# Autodesk Inventor assembly: Right Side Arm Intake
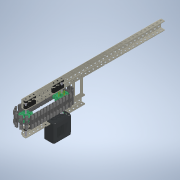
[picture p0: Inventor's stored thumbnail of the model, 180x180]
Saved by Autodesk Inventor 2020 (Build 240168000, 168)
## iProperties
Created: 2019-09-15
Part Number: Right Side Arm Intake
Document SubType Name: Assembly
Designer: Corey
Author: Corey
## Documents named in this file (10)
- C:\Users\Corey\Documents\Tower-Takeover-CAD\Parts\Right Side Arm Intake.iam
- C:\Users\Corey\Documents\Tower-Takeover-CAD\Parts\Motion\Sprockets\High Strength 12-tooth Sprocket.ipt
- C:\Users\Corey\Documents\Tower-Takeover-CAD\Parts\Structure\C-Channels\Aluminum\2-Wide\Aluminum C-Channel 1x2x1x35_MIR1.ipt
- C:\Users\Corey\Documents\Tower-Takeover-CAD\Parts\Motion\Bearing Flat_MIR4.ipt
- C:\Users\Corey\Documents\Tower-Takeover-CAD\Parts\Motion\Drive Shafts\Drive Shaft 4''_MIR1.ipt
- C:\Users\Corey\Documents\Tower-Takeover-CAD\Parts\Motion\Chain & Tank Tread\Tank Tread Traction Link_MIR1.ipt
- C:\Users\Corey\Documents\Tower-Takeover-CAD\Parts\Electronics\V5\Smart_Motor_MIR1.iam
- C:\Users\Corey\Documents\Tower-Takeover-CAD\Parts\Structure\Standoffs & Couplers\Standoff 2.00''_MIR1.ipt
- C:\Users\Corey\Documents\Tower-Takeover-CAD\Parts\Structure\C-Channels\Aluminum\2-Wide\Aluminum C-Channel 1x2x1x15_MIR1.ipt
- C:\Users\Corey\Documents\Tower-Takeover-CAD\Parts\Chain Sketch for Intake.ipt
## Components (51 placed, 9 different names)
1. Aluminum C-Channel 1x2x1x35_MIR1:1 — Insert:27, Insert:28, Mate:19, Insert:29, Insert:30, Mate:20, Insert:31, Insert:32, Mate:21, Insert:33, Insert:34, Mate:22, Insert:37, Insert:38, Mate:30, Mate:33
2. Bearing Flat_MIR4:1 — Insert:27, Insert:28, Mate:19
3. Bearing Flat_MIR4:2 — Insert:29, Insert:30, Mate:20, Insert:36
4. Bearing Flat_MIR4:3 — Insert:31, Insert:32, Mate:21
5. Bearing Flat_MIR4:4 — Insert:33, Insert:34, Mate:22, Insert:35
6. Drive Shaft 4''_MIR1:1 — Insert:35, Mate:31, Mate:32
7. Drive Shaft 4''_MIR1:2 — Insert:36, Mate:28, Mate:29
8. Smart_Motor_MIR1:1 [sub-assembly] — Insert:39, Insert:40
9. Standoff 2.00''_MIR1:1 — Insert:37, Insert:45
10. Standoff 2.00''_MIR1:2 — Insert:38, Insert:46
11. Bearing Flat_MIR4:5 — Insert:39, Insert:40, Insert:41, Insert:42
12. Bearing Flat_MIR4:6 — Insert:43, Insert:44
13. Aluminum C-Channel 1x2x1x15_MIR1:1 — Insert:41, Insert:42, Insert:43, Insert:44, Insert:45, Insert:46
14. High Strength 12-tooth Sprocket:1 — Mate:28, Mate:29, Mate:30, Flush:3
15. High Strength 12-tooth Sprocket:2 — Mate:31, Mate:32, Mate:33, Mate:34, Flush:1, Flush:2, Flush:3
16. Chain Sketch for Intake:1 — Mate:34, Flush:1, Flush:2, Flush:4, Mate:35, Mate:36
17. Tank Tread Traction Link_MIR1:1 — Flush:4, Mate:35, Mate:36
18. Tank Tread Traction Link_MIR1:2
19. Tank Tread Traction Link_MIR1:3
20. Tank Tread Traction Link_MIR1:4
21. Tank Tread Traction Link_MIR1:5
22. Tank Tread Traction Link_MIR1:6
23. Tank Tread Traction Link_MIR1:7
24. Tank Tread Traction Link_MIR1:8
25. Tank Tread Traction Link_MIR1:9
26. Tank Tread Traction Link_MIR1:10
27. Tank Tread Traction Link_MIR1:11
28. Tank Tread Traction Link_MIR1:12
29. Tank Tread Traction Link_MIR1:13
30. Tank Tread Traction Link_MIR1:14
31. Tank Tread Traction Link_MIR1:15
32. Tank Tread Traction Link_MIR1:16
33. Tank Tread Traction Link_MIR1:17
34. Tank Tread Traction Link_MIR1:18
35. Tank Tread Traction Link_MIR1:19
36. Tank Tread Traction Link_MIR1:20
37. Tank Tread Traction Link_MIR1:21
38. Tank Tread Traction Link_MIR1:22
39. Tank Tread Traction Link_MIR1:23
40. Tank Tread Traction Link_MIR1:24
41. Tank Tread Traction Link_MIR1:25
42. Tank Tread Traction Link_MIR1:26
43. Tank Tread Traction Link_MIR1:27
44. Tank Tread Traction Link_MIR1:28
45. Tank Tread Traction Link_MIR1:29
46. Tank Tread Traction Link_MIR1:30
47. Tank Tread Traction Link_MIR1:31
48. Tank Tread Traction Link_MIR1:32
49. Tank Tread Traction Link_MIR1:33
50. Tank Tread Traction Link_MIR1:34
51. Tank Tread Traction Link_MIR1:35
## Component patterns: (35 elements, first: Tank Tread Traction Link_MIR1:1)
## Relationships (37: Insert 20, Mate 13, Flush 4)
- Insert:27: Aluminum C-Channel 1x2x1x35_MIR1:1 ↔ Bearing Flat_MIR4:1
- Insert:28: Aluminum C-Channel 1x2x1x35_MIR1:1 ↔ Bearing Flat_MIR4:1
- Mate:19: Aluminum C-Channel 1x2x1x35_MIR1:1 ↔ Bearing Flat_MIR4:1
- Insert:29: Aluminum C-Channel 1x2x1x35_MIR1:1 ↔ Bearing Flat_MIR4:2
- Insert:30: Aluminum C-Channel 1x2x1x35_MIR1:1 ↔ Bearing Flat_MIR4:2
- Mate:20: Aluminum C-Channel 1x2x1x35_MIR1:1 ↔ Bearing Flat_MIR4:2
- Insert:31: Aluminum C-Channel 1x2x1x35_MIR1:1 ↔ Bearing Flat_MIR4:3
- Insert:32: Aluminum C-Channel 1x2x1x35_MIR1:1 ↔ Bearing Flat_MIR4:3
- Mate:21: Aluminum C-Channel 1x2x1x35_MIR1:1 ↔ Bearing Flat_MIR4:3
- Insert:33: Aluminum C-Channel 1x2x1x35_MIR1:1 ↔ Bearing Flat_MIR4:4
- Insert:34: Aluminum C-Channel 1x2x1x35_MIR1:1 ↔ Bearing Flat_MIR4:4
- Mate:22: Aluminum C-Channel 1x2x1x35_MIR1:1 ↔ Bearing Flat_MIR4:4
- Insert:35: Bearing Flat_MIR4:4 ↔ Drive Shaft 4''_MIR1:1
- Insert:36: Bearing Flat_MIR4:2 ↔ Drive Shaft 4''_MIR1:2
- Insert:37: Aluminum C-Channel 1x2x1x35_MIR1:1 ↔ Standoff 2.00''_MIR1:1
- Insert:38: Aluminum C-Channel 1x2x1x35_MIR1:1 ↔ Standoff 2.00''_MIR1:2
- Insert:39: Smart_Motor_MIR1:1 ↔ Bearing Flat_MIR4:5
- Insert:40: Smart_Motor_MIR1:1 ↔ Bearing Flat_MIR4:5
- Insert:41: Bearing Flat_MIR4:5 ↔ Aluminum C-Channel 1x2x1x15_MIR1:1
- Insert:42: Bearing Flat_MIR4:5 ↔ Aluminum C-Channel 1x2x1x15_MIR1:1
- Insert:43: Bearing Flat_MIR4:6 ↔ Aluminum C-Channel 1x2x1x15_MIR1:1
- Insert:44: Bearing Flat_MIR4:6 ↔ Aluminum C-Channel 1x2x1x15_MIR1:1
- Insert:45: Standoff 2.00''_MIR1:1 ↔ Aluminum C-Channel 1x2x1x15_MIR1:1
- Insert:46: Standoff 2.00''_MIR1:2 ↔ Aluminum C-Channel 1x2x1x15_MIR1:1
- Mate:28: Drive Shaft 4''_MIR1:2 ↔ High Strength 12-tooth Sprocket:1
- Mate:29: Drive Shaft 4''_MIR1:2 ↔ High Strength 12-tooth Sprocket:1
- Mate:30 (14.732 mm): Aluminum C-Channel 1x2x1x35_MIR1:1 ↔ High Strength 12-tooth Sprocket:1
- Mate:31: Drive Shaft 4''_MIR1:1 ↔ High Strength 12-tooth Sprocket:2
- Mate:32: Drive Shaft 4''_MIR1:1 ↔ High Strength 12-tooth Sprocket:2
- Mate:33 (14.732 mm): Aluminum C-Channel 1x2x1x35_MIR1:1 ↔ High Strength 12-tooth Sprocket:2
- Mate:34: High Strength 12-tooth Sprocket:2 ↔ Chain Sketch for Intake:1
- Flush:1: High Strength 12-tooth Sprocket:2 ↔ Chain Sketch for Intake:1
- Flush:2: High Strength 12-tooth Sprocket:2 ↔ Chain Sketch for Intake:1
- Flush:3: High Strength 12-tooth Sprocket:1 ↔ High Strength 12-tooth Sprocket:2
- Flush:4 (24.13 mm): Chain Sketch for Intake:1 ↔ Tank Tread Traction Link_MIR1:1
- Mate:35: Chain Sketch for Intake:1 ↔ Tank Tread Traction Link_MIR1:1
- Mate:36 (114.3 mm): Chain Sketch for Intake:1 ↔ Tank Tread Traction Link_MIR1:1
